# Autodesk Inventor assembly: Bare_Projector
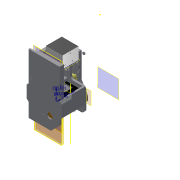
[picture p0: Inventor's stored thumbnail of the model, 180x180]
Saved by Autodesk Inventor 2016 (Build 200138000, 138)
## iProperties
Created: 2016-11-08
Part Number: Bare_Projector
Material: Generisch
Document SubType Name: Assembly
Designer: Bene
Author: Bene
## Documents named in this file (14)
- C:\Users\diederichbenedict\Documents\Inventor\Beamerscope_r4\Bare_Projector.iam
- C:\Users\diederichbenedict\Documents\Inventor\Beamerscope_r4\05_Case_Bottom.ipt
- C:\Users\diederichbenedict\Documents\Inventor\Beamerscope_r4\06_Case_Upper.ipt
- C:\Users\diederichbenedict\Documents\Inventor\Beamerscope_r4\Projector_PCB.iam
- C:\Users\diederichbenedict\Documents\Inventor\Beamerscope_r4\ACL3026U-Step.ipt
- C:\Users\diederichbenedict\Documents\Inventor\Beamerscope_r4\LED.iam
- C:\Users\diederichbenedict\Documents\Inventor\Beamerscope_r4\26_Lensholder_Aspheric_right.ipt
- C:\Users\diederichbenedict\Documents\Inventor\Beamerscope_r4\27_Nut.ipt
- C:\Users\diederichbenedict\Documents\Inventor\Beamerscope_r4\RJMP_01_08_2.ipt
- C:\Users\diederichbenedict\Documents\Inventor\Beamerscope_r4\00_Stange.ipt
- C:\Users\diederichbenedict\Documents\Inventor\Beamerscope_r4\27_Focus_Knob.ipt
- C:\Users\diederichbenedict\Documents\Inventor\Beamerscope_r4\28_Z_Stage.ipt
- C:\Users\diederichbenedict\Documents\Inventor\Beamerscope_r4\DIN EN ISO 4036 - M6.ipt
- C:\Users\diederichbenedict\Documents\Inventor\Beamerscope_r4\DIN 6912 - M6 x 20.ipt
## Components (16 placed, 13 different names)
1. 05_Case_Bottom:1 — Passend:11
2. 06_Case_Upper:1 — Fluchtend:12, Fluchtend:21, Fluchtend:22, Passend:11, Einfügen:8, Einfügen:9
3. Projector_PCB:1 [sub-assembly] — Passend:1
4. ACL3026U-Step:1 — Einfügen:1, Passend:1, Fluchtend:12
5. ACL3026U-Step:2 — Einfügen:1
6. 26_Lensholder_Aspheric_right:1
7. LED:1 [sub-assembly]
8. RJMP_01_08_2:1
9. 27_Nut:1 — Fluchtend:21, Fluchtend:22
10. 00_Stange:2 — Einfügen:9
11. 00_Stange:3 — Einfügen:8
12. RJMP_01_08_2:2
13. DIN EN ISO 4036 M6:1 — Einfügen:6
14. DIN 6912 M6 x 20:1 — Einfügen:6
15. 27_Focus_Knob:1 — Fluchtend:24
16. 28_Z_Stage:1 — Fluchtend:24
## Relationships (15: Flush 7, Insert 4, Mate 4)
- [Flush]: 05_Case_Bottom:1 ↔ Projector_PCB:1
- [Flush] (4 mm): 05_Case_Bottom:1 ↔ Projector_PCB:1
- Einfügen:1 [Insert] (-28 mm): ACL3026U-Step:1 ↔ ACL3026U-Step:2
- Passend:1 [Mate]: Projector_PCB:1 ↔ ACL3026U-Step:1
- Fluchtend:12 [Flush] (12.208 mm): 06_Case_Upper:1 ↔ ACL3026U-Step:1
- [Mate]: 06_Case_Upper:1 ↔ 26_Lensholder_Aspheric_right:1
- [Mate]: ACL3026U-Step:1 ↔ 26_Lensholder_Aspheric_right:1
- Fluchtend:21 [Flush]: 06_Case_Upper:1 ↔ 27_Nut:1
- Fluchtend:22 [Flush]: 06_Case_Upper:1 ↔ 27_Nut:1
- Passend:11 [Mate]: 05_Case_Bottom:1 ↔ 06_Case_Upper:1
- [Flush]: DIN 6912 M6 x 20:1 ↔ 27_Focus_Knob:1
- Fluchtend:24 [Flush]: 27_Focus_Knob:1 ↔ 28_Z_Stage:1
- Einfügen:6 [Insert] (6 mm): DIN EN ISO 4036 M6:1 ↔ DIN 6912 M6 x 20:1
- Einfügen:8 [Insert]: 06_Case_Upper:1 ↔ 00_Stange:3
- Einfügen:9 [Insert]: 06_Case_Upper:1 ↔ 00_Stange:2
